# Autodesk Inventor assembly: czlon3
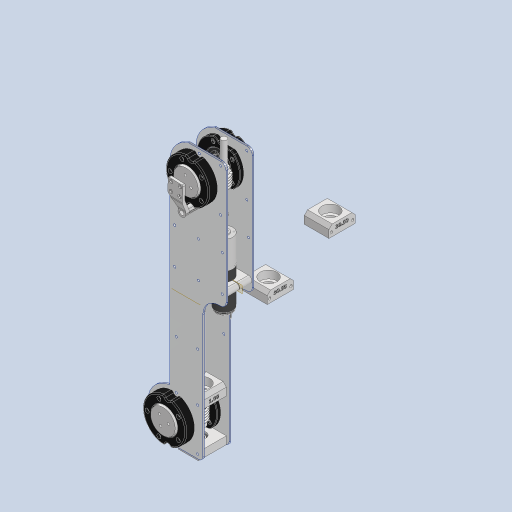
[picture p0: Inventor's stored thumbnail of the model, 512x512]
Saved by Autodesk Inventor 2023 (Build 270158000, 158)
## iProperties
Created: 2023-04-06
Part Number: czlon3
Document SubType Name: Assembly
Designer: Kamil
Author: Kamil
## Documents named in this file (18)
- C:\Users\Kamil\Desktop\KONARM_2\czlon 3\czlon3.iam
- C:\Users\Kamil\Desktop\KONARM_2\czlon 3\blacha.ipt
- C:\Users\Kamil\Desktop\KONARM_2\czlon 3\uchwyt_na_silniki_v2.ipt
- C:\Users\Kamil\Desktop\KONARM_2\czlon 3\kolnierz wewnetrzny.ipt
- C:\Users\Kamil\Desktop\KONARM_2\czlon 3\koszyczek.ipt
- C:\Users\Kamil\Desktop\KONARM_2\czlon 3\staw.iam
- C:\Users\Kamil\Desktop\KONARM_2\czlon 3\Faulhaber 3272G012C R.ipt
- C:\Users\Kamil\Desktop\KONARM_2\czlon 3\wał_2.ipt
- C:\Users\Kamil\Desktop\KONARM_2\czlon 3\os_napedowa.ipt
- C:\Users\Kamil\Desktop\KONARM_2\czlon 3\Złożenie2.STEP.ipt
- C:\Users\Kamil\Desktop\KONARM_2\czlon 3\blacha_MIR.ipt
- C:\Users\Kamil\Desktop\KONARM_2\czlon 3\kolnierz wewnetrzny_MIR.ipt
- C:\Users\Kamil\Desktop\KONARM_2\czlon 3\koszyczek_MIR.ipt
- C:\Users\Kamil\Desktop\KONARM_2\czlon 3\Uchwyt_na_enkoder.ipt
- C:\Users\Kamil\Documents\Inventor\Konarm\uchwyt_na_sil.ipt
- C:\Users\Kamil\Desktop\KONARM_2\czlon 3\uchwyt_lozyska\uchwyt_lozyska_1mm.ipt
- C:\Users\Kamil\Desktop\KONARM_2\czlon 3\uchwyt_lozyska.ipt
- C:\Users\Kamil\Desktop\KONARM_2\czlon 3\3200_2rs.ipt
## Components (28 placed, 16 different names)
1. blacha:1 — Zestawiające:1, Zestawiające:2, Zestawiające:3, Zestawiające:7, Zestawiające:8, Zestawiające:9, Zestawiające:10, Zestawiające:11, Zestawiające:12, Zestawiające:13, Zestawiające:14, Zestawiające:15, Zestawiające:16, Zestawiające:17, Zestawiające:18, Zestawiające:19, Zestawiające:20, Zestawiające:21, Zestawiające:22, Zestawiające:50, Zestawiające:51, Zestawiające:54, Zestawiające:56
2. uchwyt_na_silniki_v2:1 — Zestawiające:1, Zestawiające:2, Zestawiające:3, Zestawiające:23, Zestawiające:24, Zestawiające:34, Symetria:1
3. kolnierz wewnetrzny:1 — Zestawiające:7, Zestawiające:9, Zestawiające:11
4. kolnierz wewnetrzny:2 — Zestawiające:8, Zestawiające:10, Zestawiające:12
5. koszyczek:1 — Zestawiające:18, Zestawiające:21, Zestawiające:22
6. koszyczek:2 — Zestawiające:17, Zestawiające:19, Zestawiające:20
7. staw:1 [sub-assembly] — Zestawiające:15, Zestawiające:16, Zestawiające:32
8. staw:2 [sub-assembly] — Zestawiające:13, Zestawiające:14, Zestawiające:30
9. Faulhaber 3272G012C R:1 — Zestawiające:24, Zestawiające:28
10. Faulhaber 3272G012C R:2 — Zestawiające:23, Zestawiające:26, Zestawiające:33
11. wał_2:1 — Zestawiające:28, Zestawiające:29
12. os_napedowa:1 — Zestawiające:26, Zestawiające:31, Zestawiające:57
13. Złożenie2.STEP:1 — Zestawiające:29, Zestawiające:30
14. Złożenie2.STEP:2 — Zestawiające:31, Zestawiające:32
15. uchwyt_na_silniki_v2:2 — Zestawiające:33, Zestawiające:34, Symetria:1
16. blacha_MIR:1 — Zestawiające:36, Zestawiające:37, Zestawiające:38, Zestawiające:39, Zestawiające:40, Zestawiające:41, Zestawiające:42, Zestawiające:43, Zestawiające:44, Zestawiające:45, Zestawiające:46, Zestawiające:47, Zestawiające:48, Zestawiające:49, Równoległe:1, Równoległe:2, Zestawiające:52, Zestawiające:53, Zestawiające:55
17. kolnierz wewnetrzny_MIR:1 — Zestawiające:36, Zestawiające:37, Zestawiające:38
18. kolnierz wewnetrzny_MIR:2 — Zestawiające:39, Zestawiające:40, Zestawiające:41
19. koszyczek_MIR:1 — Zestawiające:42, Zestawiające:43, Zestawiające:44
20. koszyczek_MIR:2 — Zestawiające:45, Zestawiające:46, Zestawiające:47
21. Uchwyt_na_enkoder:3 — Zestawiające:48, Zestawiające:49
22. Uchwyt_na_enkoder:4 — Zestawiające:50, Zestawiające:51
23. uchwyt_na_sil:1 — Równoległe:1, Równoległe:2
24. uchwyt_lozyska_1mm:1
25. uchwyt_lozyska_1mm:2
26. uchwyt_lozyska_1mm:3 — Zestawiające:55, Zestawiające:56
27. uchwyt_lozyska_1mm:4 — Zestawiające:52, Zestawiające:53, Zestawiające:54
28. 3200_2rs:1 — Zestawiające:57
## Relationships (54: Mate 51, Flush 2, Symmetry 1)
- Zestawiające:1 [Mate]: blacha:1 ↔ uchwyt_na_silniki_v2:1
- Zestawiające:2 [Mate]: blacha:1 ↔ uchwyt_na_silniki_v2:1
- Zestawiające:3 [Mate]: blacha:1 ↔ uchwyt_na_silniki_v2:1
- Zestawiające:7 [Mate]: blacha:1 ↔ kolnierz wewnetrzny:1
- Zestawiające:8 [Mate]: blacha:1 ↔ kolnierz wewnetrzny:2
- Zestawiające:9 [Mate]: blacha:1 ↔ kolnierz wewnetrzny:1
- Zestawiające:10 [Mate]: blacha:1 ↔ kolnierz wewnetrzny:2
- Zestawiające:11 [Mate]: blacha:1 ↔ kolnierz wewnetrzny:1
- Zestawiające:12 [Mate]: blacha:1 ↔ kolnierz wewnetrzny:2
- Zestawiające:13 [Mate]: blacha:1 ↔ staw:2
- Zestawiające:14 [Mate]: blacha:1 ↔ staw:2
- Zestawiające:15 [Mate]: blacha:1 ↔ staw:1
- Zestawiające:16 [Mate]: blacha:1 ↔ staw:1
- Zestawiające:17 [Mate]: blacha:1 ↔ koszyczek:2
- Zestawiające:18 [Mate]: blacha:1 ↔ koszyczek:1
- Zestawiające:19 [Mate]: blacha:1 ↔ koszyczek:2
- Zestawiające:20 [Mate]: blacha:1 ↔ koszyczek:2
- Zestawiające:21 [Mate]: blacha:1 ↔ koszyczek:1
- Zestawiające:22 [Mate]: blacha:1 ↔ koszyczek:1
- Zestawiające:23 [Mate]: uchwyt_na_silniki_v2:1 ↔ Faulhaber 3272G012C R:2
- Zestawiające:24 [Mate]: uchwyt_na_silniki_v2:1 ↔ Faulhaber 3272G012C R:1
- Zestawiające:26 [Mate]: Faulhaber 3272G012C R:2 ↔ os_napedowa:1
- Zestawiające:28 [Mate]: Faulhaber 3272G012C R:1 ↔ wał_2:1
- Zestawiające:29 [Mate]: wał_2:1 ↔ Złożenie2.STEP:1
- Zestawiające:30 [Mate]: staw:2 ↔ Złożenie2.STEP:1
- Zestawiające:31 [Mate]: os_napedowa:1 ↔ Złożenie2.STEP:2
- Zestawiające:32 [Mate]: staw:1 ↔ Złożenie2.STEP:2
- Zestawiające:33 [Mate]: Faulhaber 3272G012C R:2 ↔ uchwyt_na_silniki_v2:2
- Zestawiające:34 [Mate]: uchwyt_na_silniki_v2:1 ↔ uchwyt_na_silniki_v2:2
- Symetria:1 [Symmetry]: uchwyt_na_silniki_v2:1 ↔ uchwyt_na_silniki_v2:2
- Zestawiające:36 [Mate]: blacha_MIR:1 ↔ kolnierz wewnetrzny_MIR:1
- Zestawiające:37 [Mate]: blacha_MIR:1 ↔ kolnierz wewnetrzny_MIR:1
- Zestawiające:38 [Mate]: blacha_MIR:1 ↔ kolnierz wewnetrzny_MIR:1
- Zestawiające:39 [Mate]: blacha_MIR:1 ↔ kolnierz wewnetrzny_MIR:2
- Zestawiające:40 [Mate]: blacha_MIR:1 ↔ kolnierz wewnetrzny_MIR:2
- Zestawiające:41 [Mate]: blacha_MIR:1 ↔ kolnierz wewnetrzny_MIR:2
- Zestawiające:42 [Mate]: blacha_MIR:1 ↔ koszyczek_MIR:1
- Zestawiające:43 [Mate]: blacha_MIR:1 ↔ koszyczek_MIR:1
- Zestawiające:44 [Mate]: blacha_MIR:1 ↔ koszyczek_MIR:1
- Zestawiające:45 [Mate]: blacha_MIR:1 ↔ koszyczek_MIR:2
- Zestawiające:46 [Mate]: blacha_MIR:1 ↔ koszyczek_MIR:2
- Zestawiające:47 [Mate]: blacha_MIR:1 ↔ koszyczek_MIR:2
- Zestawiające:48 [Mate]: blacha_MIR:1 ↔ Uchwyt_na_enkoder:3
- Zestawiające:49 [Mate]: blacha_MIR:1 ↔ Uchwyt_na_enkoder:3
- Zestawiające:50 [Mate]: blacha:1 ↔ Uchwyt_na_enkoder:4
- Zestawiające:51 [Mate]: blacha:1 ↔ Uchwyt_na_enkoder:4
- Równoległe:1 [Flush]: blacha_MIR:1 ↔ uchwyt_na_sil:1
- Równoległe:2 [Flush]: blacha_MIR:1 ↔ uchwyt_na_sil:1
- Zestawiające:52 [Mate]: blacha_MIR:1 ↔ uchwyt_lozyska_1mm:4
- Zestawiające:53 [Mate]: blacha_MIR:1 ↔ uchwyt_lozyska_1mm:4
- Zestawiające:54 [Mate]: blacha:1 ↔ uchwyt_lozyska_1mm:4
- Zestawiające:55 [Mate]: blacha_MIR:1 ↔ uchwyt_lozyska_1mm:3
- Zestawiające:56 [Mate]: blacha:1 ↔ uchwyt_lozyska_1mm:3
- Zestawiające:57 [Mate]: os_napedowa:1 ↔ 3200_2rs:1
